# Autodesk Inventor assembly: Chessboard Hardware Model
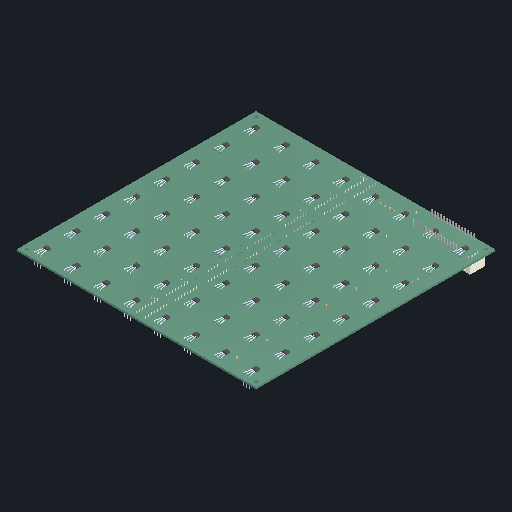
[picture p0: Inventor's stored thumbnail of the model, 512x512]
Saved by Autodesk Inventor 2026 (Build 300175000, 175)
## iProperties
Created: 2025-04-15
Part Number: Chessboard Hardware Model
Document SubType Name: Assembly
Designer: ckyiu
Author: ckyiu
## iProperties of the stored document Chessboard Hardware Model.iam
Created: 2025-03-10
Part Number: Chessboard Hardware Model
Description: KiCad electronic assembly
Document SubType Name: Assembly
Designer: ckyiu
Sending System: Autodesk Translation Framework v13.20.0.188
Preprocessor: ST-DEVELOPER v20
Title: Chessboard Hardware Model v1.step
## iProperties of the stored document PinHeader_1x01_P2.54mm_Vertical.iam
Created: 2025-04-15
Part Number: PinHeader_1x01_P2.54mm_Vertical
Document SubType Name: Assembly
Designer: ckyiu
Author: ckyiu
## iProperties of the stored document Arduino Nano v10 (1).iam
Created: 2025-04-15
Part Number: Arduino Nano v10
Document SubType Name: Assembly
Designer: ckyiu
Author: ckyiu
## iProperties of the stored document C_Disc_D50mm_W25mm_P250mm.ipt
Created: 2025-04-15
Part Number: C_Disc_D50mm_W25mm_P250mm
Material: Steel
Document SubType Name: Modeling
Designer: ckyiu
Density: 7.85 g/cm^3
Appearance: Default
Author: ckyiu
## iProperties of the stored document C_Disc_D5.0mm_W2.5mm_P2.50mm.iam
Created: 2025-04-15
Part Number: C_Disc_D5.0mm_W2.5mm_P2.50mm
Document SubType Name: Assembly
Designer: ckyiu
Author: ckyiu
## iProperties of the stored document JST_XH_B4B-XH-A_1x04_P2.50mm_Vertical.iam
Created: 2025-04-15
Part Number: JST_XH_B4B-XH-A_1x04_P2.50mm_Vertical
Document SubType Name: Assembly
Designer: ckyiu
Author: ckyiu
## iProperties of the stored document _autosave-Chessboard Hardware_PCB.ipt
Created: 2025-04-15
Part Number: _autosave-Chessboard Hardware_PCB
Material: Steel
Document SubType Name: Modeling
Designer: ckyiu
Density: 7.85 g/cm^3
Appearance: Default
Author: ckyiu
## iProperties of the stored document DIP-16_W7.62mm (1).iam
Created: 2025-04-15
Part Number: DIP-16_W7.62mm
Document SubType Name: Assembly
Designer: ckyiu
Author: ckyiu
## iProperties of the stored document PinHeader_1x01_P254mm_Vertical.ipt
Created: 2025-04-15
Part Number: PinHeader_1x01_P254mm_Vertical
Material: Steel
Document SubType Name: Modeling
Designer: ckyiu
Density: 7.85 g/cm^3
Appearance: Default
Author: ckyiu
## iProperties of the stored document SS49E lay flat v10 (1).iam
Created: 2025-04-15
Part Number: SS49E lay flat v10
Document SubType Name: Assembly
Designer: ckyiu
Author: ckyiu
## iProperties of the stored document DIP-16_W7.62mm.ipt
Created: 2025-04-15
Part Number: DIP-16_W7.62mm_1
Material: Steel
Document SubType Name: Modeling
Designer: ckyiu
Density: 7.85 g/cm^3
Appearance: Default
Author: ckyiu
## iProperties of the stored document Arduino Nano v10.ipt
Created: 2025-04-15
Part Number: Arduino Nano v10_1
Material: Steel
Document SubType Name: Modeling
Designer: ckyiu
Density: 7.85 g/cm^3
Appearance: Default
Author: ckyiu
## iProperties of the stored document SS49E lay flat v10.ipt
Created: 2025-04-15
Part Number: SS49E lay flat v10_1
Material: Steel
Document SubType Name: Modeling
Designer: ckyiu
Density: 7.85 g/cm^3
Appearance: Default
Author: ckyiu
## iProperties of the stored document JST_B4B_XH_A.ipt
Created: 2025-04-15
Part Number: JST_B4B_XH_A
Material: Steel
Document SubType Name: Modeling
Designer: ckyiu
Density: 7.85 g/cm^3
Appearance: Default
Author: ckyiu
## Documents named in this file (17)
- F:\Chessboard-Design\Assemblies\PCBs\Chessboard Hardware Model.iam
- **F:\Chessboard-Design\Assemblies\PCBs\Chessboard Hardware Model.iam*LocalDocs*xAaaaanaaAaaaaaaaAaaaqmdb4e*Chessboard Hardware Model.iam
- **C:\Users\ckyiu\Documents\Projects\Chessboard-Design\Assemblies\PCBs\Chessboard Hardware Model.iam*LocalDocs*xAaaaanaaAaaaaaaaAaaaqmdb4e*Chessboard Hardware Model.iam
- **C:\Users\ckyiu\Documents\Projects\Chessboard-Design\Assemblies\PCBs\Chessboard Hardware Model.iam*LocalDocs*xAaaaqjcaAaaaaaaaAaaaqsxoMh*SS49E lay flat v10 (1).iam
- **C:\Users\ckyiu\Documents\Projects\Chessboard-Design\Assemblies\PCBs\Chessboard Hardware Model.iam*LocalDocs*xAaaaqecaAaaaaaaaAaaaa4vkWa*DIP-16_W7.62mm (1).iam
- **C:\Users\ckyiu\Documents\Projects\Chessboard-Design\Assemblies\PCBs\Chessboard Hardware Model.iam*LocalDocs*xAaaaaecaAaaaaaaaAaaaqpubQd*PinHeader_1x01_P2.54mm_Vertical.iam
- **C:\Users\ckyiu\Documents\Projects\Chessboard-Design\Assemblies\PCBs\Chessboard Hardware Model.iam*LocalDocs*xAaaaqgcaAaaaaaaaAaaaq2dwKg*C_Disc_D5.0mm_W2.5mm_P2.50mm.iam
- **C:\Users\ckyiu\Documents\Projects\Chessboard-Design\Assemblies\PCBs\Chessboard Hardware Model.iam*LocalDocs*xAaaaacbaAaaaaaaaAaaaav5n3g*Arduino Nano v10 (1).iam
- **C:\Users\ckyiu\Documents\Projects\Chessboard-Design\Assemblies\PCBs\Chessboard Hardware Model.iam*LocalDocs*xAaaaazaaAaaaaaaaAaaaarowPd*JST_XH_B4B-XH-A_1x04_P2.50mm_Vertical.iam
- **C:\Users\ckyiu\Documents\Projects\Chessboard-Design\Assemblies\PCBs\Chessboard Hardware Model.iam*LocalDocs*xAaaaarcaAaaaaaaaAaaaqlz0Ye*_autosave-Chessboard Hardware_PCB.ipt
- **C:\Users\ckyiu\Documents\Projects\Chessboard-Design\Assemblies\PCBs\Chessboard Hardware Model.iam*LocalDocs*xAaaaqkcaAaaaaaaaAaaaaruiCe*PinHeader_1x01_P254mm_Vertical.ipt
- **C:\Users\ckyiu\Documents\Projects\Chessboard-Design\Assemblies\PCBs\Chessboard Hardware Model.iam*LocalDocs*xAaaaqnaaAaaaaaaaAaaaqwodVe*Arduino Nano v10.ipt
- **C:\Users\ckyiu\Documents\Projects\Chessboard-Design\Assemblies\PCBs\Chessboard Hardware Model.iam*LocalDocs*xAaaaalbaAaaaaaaaAaaaqitwAh*C_Disc_D50mm_W25mm_P250mm.ipt
- **C:\Users\ckyiu\Documents\Projects\Chessboard-Design\Assemblies\PCBs\Chessboard Hardware Model.iam*LocalDocs*xAaaaqxdaAaaaaaaaAaaaqklxJh*JST_B4B_XH_A.ipt
- **C:\Users\ckyiu\Documents\Projects\Chessboard-Design\Assemblies\PCBs\Chessboard Hardware Model.iam*LocalDocs*xAaaaqpaaAaaaaaaaAaaaqb4eOd*DIP-16_W7.62mm.ipt
- **C:\Users\ckyiu\Documents\Projects\Chessboard-Design\Assemblies\PCBs\Chessboard Hardware Model.iam*LocalDocs*xAaaaqpcaAaaaaaaaAaaaay3oUd*SS49E lay flat v10.ipt
- F:\Chessboard-Design\Assemblies\PCBs\Chessboard Hardware Model.step
## Components (1 placed, 1 different names)
1. Chessboard Hardware Model:1 [sub-assembly] — Mate:1, Mate:2, Mate:3
## Relationships (3: Mate 3)
- Mate:1 (-100 mm): Chessboard Hardware Model:1
- Mate:2 (-100 mm): Chessboard Hardware Model:1
- Mate:3: Chessboard Hardware Model:1
